# Autodesk Inventor assembly: Assembly1
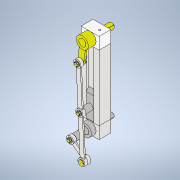
[picture p0: Inventor's stored thumbnail of the model, 180x180]
Saved by Autodesk Inventor 2020.5 (Build 245400000, 400)
## iProperties
Created: 2020-07-24
Part Number: Assembly1
Document SubType Name: Assembly
Designer: admin
Author: admin
## Documents named in this file (11)
- C:\Users\André Aguirre Apolo\Desktop\ESPOL\PAO2, 2022\Diseño y simulacion de maquinas\Teorico\proyecto\Assembly1.iam
- C:\Users\André Aguirre Apolo\Desktop\ESPOL\PAO2, 2022\Diseño y simulacion de maquinas\Teorico\proyecto\Bearing.ipt
- C:\Users\André Aguirre Apolo\Desktop\ESPOL\PAO2, 2022\Diseño y simulacion de maquinas\Teorico\proyecto\Crank1.ipt
- C:\Users\André Aguirre Apolo\Desktop\ESPOL\PAO2, 2022\Diseño y simulacion de maquinas\Teorico\proyecto\Conrod3.ipt
- C:\Users\André Aguirre Apolo\Desktop\ESPOL\PAO2, 2022\Diseño y simulacion de maquinas\Teorico\proyecto\Slider.ipt
- C:\Users\André Aguirre Apolo\Desktop\ESPOL\PAO2, 2022\Diseño y simulacion de maquinas\Teorico\proyecto\Conrod2.ipt
- C:\Users\André Aguirre Apolo\Desktop\ESPOL\PAO2, 2022\Diseño y simulacion de maquinas\Teorico\proyecto\Runway.ipt
- C:\Users\André Aguirre Apolo\Desktop\ESPOL\PAO2, 2022\Diseño y simulacion de maquinas\Teorico\proyecto\Crank2.ipt
- C:\Users\André Aguirre Apolo\Desktop\ESPOL\PAO2, 2022\Diseño y simulacion de maquinas\Teorico\proyecto\Pin.ipt
- C:\Users\André Aguirre Apolo\Desktop\ESPOL\PAO2, 2022\Diseño y simulacion de maquinas\Teorico\proyecto\Pin610.ipt
- C:\Users\André Aguirre Apolo\Desktop\ESPOL\PAO2, 2022\Diseño y simulacion de maquinas\Teorico\proyecto\Bolt3W.ipt
## Components (14 placed, 10 different names)
1. Runway:1 — Coincidencia:1
2. Pin:1
3. Pin:2
4. Bearing:2 — Flush:1, Flush:2, Flush:3, Insert:2
5. Bearing:1 — Flush:1, Flush:2, Flush:3, Insert:6
6. Crank2:1 — Insert:3, Insert:6, Insert:12
7. Crank1:2 — Insert:2, Insert:5, Insert:10
8. Conrod3:1 — Insert:3, Insert:4, Insertar:13
9. Slider:1 — Insert:4, Insert:11, Coincidencia:1
10. Conrod2:1 — Insert:5, Insert:9, Insertar:13
11. Pin610:1 — Insert:9
12. Bolt3W:1 — Insert:12
13. Bolt3W:2 — Insert:11
14. Bolt3W:3 — Insert:10
## Relationships (14: Insert 10, Flush 3, Mate 1)
- Flush:1: Bearing:2 ↔ Bearing:1
- Flush:2: Bearing:2 ↔ Bearing:1
- Flush:3 (-130 mm): Bearing:2 ↔ Bearing:1
- Insert:2: Bearing:2 ↔ Crank1:2
- Insert:3: Crank2:1 ↔ Conrod3:1
- Insert:4: Conrod3:1 ↔ Slider:1
- Insert:5: Crank1:2 ↔ Conrod2:1
- Insert:6: Bearing:1 ↔ Crank2:1
- Insert:9: Conrod2:1 ↔ Pin610:1
- Insert:10: Crank1:2 ↔ Bolt3W:3
- Insert:11: Slider:1 ↔ Bolt3W:2
- Insert:12: Crank2:1 ↔ Bolt3W:1
- Insertar:13: Conrod3:1 ↔ Conrod2:1
- Coincidencia:1 [Mate]: Runway:1 ↔ Slider:1
